# Autodesk Inventor assembly: polulu_caster_assembly
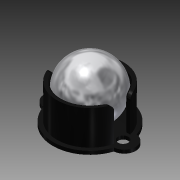
[picture p0: Inventor's stored thumbnail of the model, 180x180]
Saved by Autodesk Inventor 2014 (Build 180170000, 170)
## iProperties
Created: 2015-05-04
Part Number: polulu_caster_assembly
Document SubType Name: Assembly
Designer: Gabriel
Author: Gabriel
## Documents named in this file (3)
- C:\Users\Gabriel\Desktop\Esboço_robô\polulu_caster_assembly.iam
- C:\Users\Gabriel\Desktop\Esboço_robô\polulu_caster.ipt
- C:\Users\Gabriel\Desktop\Esboço_robô\caster_ball.ipt
## Components (2 placed, 2 different names)
1. polulu_caster:1 — Cylindrical:1
2. caster_ball:1 — Cylindrical:1
## Relationships (1: CylindricalJoint 1)
- Cylindrical:1: polulu_caster:1 ↔ caster_ball:1
